# Autodesk Inventor assembly: axe_codeur
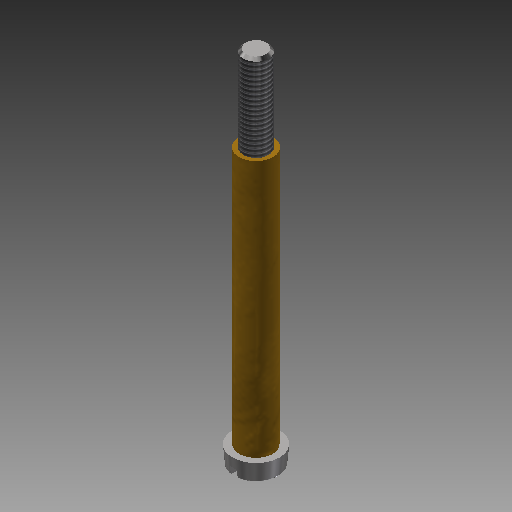
[picture p0: Inventor's stored thumbnail of the model, 512x512]
Saved by Autodesk Inventor 2019 (Build 230136000, 136)
## iProperties
Created: 2017-12-27
Part Number: axe_codeur
Document SubType Name: Assembly
Designer: franc
Mass: 2.47705 g
Surface Area: 11.1316 cm^2
Volume: 0.459471 cm^3
Density: 5.39109 g/cm^3
Author: franc
## Documents named in this file (3)
- C:\Users\franc\Desktop\EsialRobotik\Mecanique\base_roulante\axe_codeur.iam
- C:\Users\franc\Desktop\EsialRobotik\Mecanique\base_roulante\tube_laiton.ipt
- C:\Users\franc\Desktop\EsialRobotik\Mecanique\Content Center Files\R2017\fr-FR\CNS 4355\CNS 4355 - M 3 x 40.ipt
## Components (2 placed, 2 different names)
1. tube_laiton:1 — Placage:1, Placage:2
2. CNS 4355 M 3 x 40:1 — Placage:1, Placage:2
## Relationships (2: Mate 2)
- Placage:1 [Mate]: tube_laiton:1 ↔ CNS 4355 M 3 x 40:1
- Placage:2 [Mate]: tube_laiton:1 ↔ CNS 4355 M 3 x 40:1
